# Autodesk Inventor assembly: screen
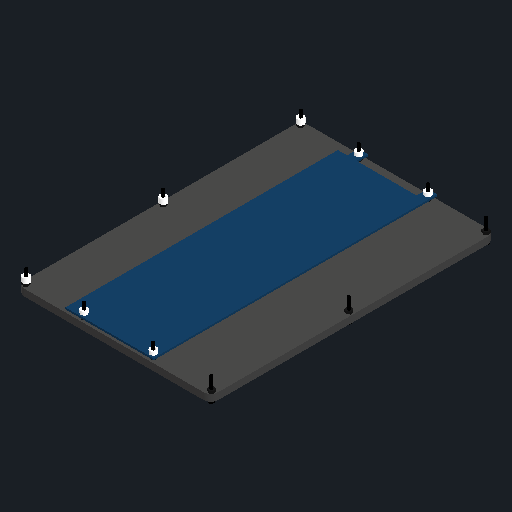
[picture p0: Inventor's stored thumbnail of the model, 512x512]
Saved by Autodesk Inventor 2026.2 (Build 302298000, 298)
## iProperties
Created: 2026-01-27
Part Number: screen
Document SubType Name: Assembly
Designer: test
Author: test
## Documents named in this file (7)
- C:\Users\test\Projects\simple-concert-monitor\simple-concert-monitor_Mechanical\screen\screen.iam
- C:\Users\test\Projects\simple-concert-monitor\simple-concert-monitor_Mechanical\screen\pcb.ipt
- C:\Users\test\Projects\simple-concert-monitor\simple-concert-monitor_Mechanical\screen\screen_module.ipt
- C:\Users\test\Projects\simple-concert-monitor\simple-concert-monitor_Mechanical\screen\screw.ipt
- C:\Users\test\Projects\simple-concert-monitor\simple-concert-monitor_Mechanical\screen\nut.ipt
- C:\Users\test\Projects\simple-concert-monitor\simple-concert-monitor_Mechanical\screen\distance_big.ipt
- C:\Users\test\Projects\simple-concert-monitor\simple-concert-monitor_Mechanical\screen\distance_small.ipt
## Components (29 placed, 6 different names)
1. pcb:1 — Mate:1, Mate:2, Mate:42, Mate:50, Mate:54, Mate:55, Mate:56
2. screen_module:1 — Mate:1, Mate:2, Mate:3, Mate:4, Mate:5, Mate:6, Mate:7, Mate:8, Mate:9, Mate:10, Mate:11, Mate:12, Mate:13, Mate:14, Mate:15, Mate:16, Mate:17, Mate:18, Mate:19, Mate:20, Mate:21, Mate:22, Mate:33, Mate:34, Mate:35, Mate:36, Mate:37, Mate:38, Mate:39, Mate:40, Mate:41
3. screw:1 — Mate:3, Mate:14, Mate:28, Mate:43
4. nut:1 — Mate:23, Mate:41
5. screw:2 — Mate:4, Mate:22, Mate:29, Mate:44
6. screw:3 — Mate:5, Mate:21, Mate:30, Mate:51
7. screw:4 — Mate:6, Mate:20, Mate:31
8. screw:5 — Mate:7, Mate:19, Mate:32
9. screw:6 — Mate:8, Mate:18, Mate:23
10. screw:7 — Mate:9, Mate:17, Mate:24, Mate:52
11. screw:8 — Mate:10, Mate:16, Mate:25, Mate:53
12. screw:9 — Mate:11, Mate:15, Mate:26, Mate:46
13. screw:10 — Mate:12, Mate:13, Mate:27, Mate:45
14. nut:2 — Mate:32, Mate:33
15. nut:3 — Mate:31, Mate:34
16. nut:4 — Mate:30, Mate:35, Mate:42
17. nut:5 — Mate:29
18. nut:6 — Mate:28, Mate:36, Mate:49
19. nut:7 — Mate:27, Mate:37, Mate:48
20. nut:8 — Mate:26, Mate:38, Mate:47
21. nut:9 — Mate:25, Mate:39
22. nut:10 — Mate:24, Mate:40
23. distance_big:1 — Mate:43, Mate:49
24. distance_small:1 — Mate:44, Mate:50
25. distance_big:2 — Mate:45, Mate:48
26. distance_big:3 — Mate:46, Mate:47
27. distance_small:2 — Mate:51, Mate:56
28. distance_small:3 — Mate:52, Mate:55
29. distance_small:4 — Mate:53, Mate:54
## Relationships (56: Mate 56)
- Mate:1: pcb:1 ↔ screen_module:1
- Mate:2: pcb:1 ↔ screen_module:1
- Mate:3: screen_module:1 ↔ screw:1
- Mate:4: screen_module:1 ↔ screw:2
- Mate:5: screen_module:1 ↔ screw:3
- Mate:6: screen_module:1 ↔ screw:4
- Mate:7: screen_module:1 ↔ screw:5
- Mate:8: screen_module:1 ↔ screw:6
- Mate:9: screen_module:1 ↔ screw:7
- Mate:10: screen_module:1 ↔ screw:8
- Mate:11: screen_module:1 ↔ screw:9
- Mate:12: screen_module:1 ↔ screw:10
- Mate:13: screen_module:1 ↔ screw:10
- Mate:14: screen_module:1 ↔ screw:1
- Mate:15: screen_module:1 ↔ screw:9
- Mate:16: screen_module:1 ↔ screw:8
- Mate:17: screen_module:1 ↔ screw:7
- Mate:18: screen_module:1 ↔ screw:6
- Mate:19: screen_module:1 ↔ screw:5
- Mate:20: screen_module:1 ↔ screw:4
- Mate:21: screen_module:1 ↔ screw:3
- Mate:22: screen_module:1 ↔ screw:2
- Mate:23: nut:1 ↔ screw:6
- Mate:24: screw:7 ↔ nut:10
- Mate:25: screw:8 ↔ nut:9
- Mate:26: screw:9 ↔ nut:8
- Mate:27: screw:10 ↔ nut:7
- Mate:28: screw:1 ↔ nut:6
- Mate:29: screw:2 ↔ nut:5
- Mate:30: screw:3 ↔ nut:4
- Mate:31: screw:4 ↔ nut:3
- Mate:32: screw:5 ↔ nut:2
- Mate:33: screen_module:1 ↔ nut:2
- Mate:34: screen_module:1 ↔ nut:3
- Mate:35: screen_module:1 ↔ nut:4
- Mate:36: screen_module:1 ↔ nut:6
- Mate:37: screen_module:1 ↔ nut:7
- Mate:38: screen_module:1 ↔ nut:8
- Mate:39: screen_module:1 ↔ nut:9
- Mate:40: screen_module:1 ↔ nut:10
- Mate:41: screen_module:1 ↔ nut:1
- Mate:42: pcb:1 ↔ nut:4
- Mate:43: screw:1 ↔ distance_big:1
- Mate:44: screw:2 ↔ distance_small:1
- Mate:45: screw:10 ↔ distance_big:2
- Mate:46: screw:9 ↔ distance_big:3
- Mate:47: nut:8 ↔ distance_big:3
- Mate:48: nut:7 ↔ distance_big:2
- Mate:49: nut:6 ↔ distance_big:1
- Mate:50: pcb:1 ↔ distance_small:1
- Mate:51: screw:3 ↔ distance_small:2
- Mate:52: screw:7 ↔ distance_small:3
- Mate:53: screw:8 ↔ distance_small:4
- Mate:54: pcb:1 ↔ distance_small:4
- Mate:55: pcb:1 ↔ distance_small:3
- Mate:56: pcb:1 ↔ distance_small:2
